# Autodesk Inventor assembly: mainflap_side
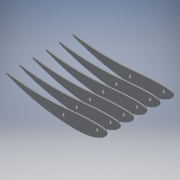
[picture p0: Inventor's stored thumbnail of the model, 180x180]
Saved by Autodesk Inventor 2018.2 (Build 222227000, 227)
## iProperties
Created: 2018-03-05
Part Number: mainflap_side
Material: 一般
Document SubType Name: Assembly
Designer: ku_sk
Author: ku_sk
## Documents named in this file (2)
- C:\Users\ku_sk\Documents\Inventor\AeroCAD2018\設計\Fr.wing\製作用\parts\mainflap_side\mainflap_side.iam
- C:\Users\ku_sk\Documents\Inventor\AeroCAD2018\設計\Fr.wing\製作用\parts\mainflap_side\plate_ms.ipt
## Components (6 placed, 1 different names)
1. plate_ms:1 — フラッシュ:1, メイト:2, メイト:3, メイト:13, メイト:22
2. plate_ms:2 — メイト:1, メイト:2, メイト:3, メイト:4, フラッシュ:2, メイト:5, メイト:14
3. plate_ms:3 — フラッシュ:2, フラッシュ:3, メイト:5, メイト:6, メイト:14, メイト:15
4. plate_ms:4 — フラッシュ:3, メイト:6, メイト:15, フラッシュ:10
5. plate_ms:9 — フラッシュ:9, メイト:12, メイト:21, フラッシュ:10
6. plate_ms:10 — フラッシュ:9, メイト:12, メイト:13, メイト:21, メイト:22
## Relationships (17: Mate 12, Flush 5)
- フラッシュ:1 [Flush] (-110 mm): plate_ms:1
- メイト:1 [Mate] (-110 mm): plate_ms:2
- メイト:2 [Mate]: plate_ms:1 ↔ plate_ms:2
- メイト:3 [Mate]: plate_ms:1 ↔ plate_ms:2
- メイト:4 [Mate]: plate_ms:2
- フラッシュ:2 [Flush] (-43 mm): plate_ms:2 ↔ plate_ms:3
- フラッシュ:3 [Flush] (-43 mm): plate_ms:3 ↔ plate_ms:4
- フラッシュ:9 [Flush] (-43 mm): plate_ms:9 ↔ plate_ms:10
- メイト:5 [Mate]: plate_ms:2 ↔ plate_ms:3
- メイト:6 [Mate]: plate_ms:3 ↔ plate_ms:4
- メイト:12 [Mate]: plate_ms:9 ↔ plate_ms:10
- メイト:13 [Mate]: plate_ms:1 ↔ plate_ms:10
- メイト:14 [Mate]: plate_ms:2 ↔ plate_ms:3
- メイト:15 [Mate]: plate_ms:3 ↔ plate_ms:4
- メイト:21 [Mate]: plate_ms:9 ↔ plate_ms:10
- メイト:22 [Mate]: plate_ms:1 ↔ plate_ms:10
- フラッシュ:10 [Flush] (-43 mm): plate_ms:4 ↔ plate_ms:9
